# Autodesk Inventor assembly: Finishing_assembly
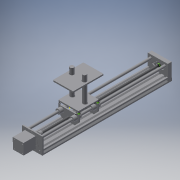
[picture p0: Inventor's stored thumbnail of the model, 180x180]
Saved by Autodesk Inventor 2019 (Build 230136000, 136)
## iProperties
Created: 2021-06-25
Part Number: Finishing_assembly
Document SubType Name: Assembly
Designer: 91742
Author: 91742
## Documents named in this file (17)
- C:\Users\91742\3D Objects\Finishing_assembly.iam
- C:\Users\91742\3D Objects\Rail_finished.ipt
- C:\Users\91742\3D Objects\Stepper_to_rail.ipt
- C:\Users\91742\3D Objects\End_atrail.ipt
- C:\Users\91742\3D Objects\Ball Baering.ipt
- C:\Users\91742\3D Objects\Dampner.ipt
- C:\Users\91742\3D Objects\Motor.ipt
- C:\Users\91742\3D Objects\Coupler.ipt
- C:\Users\91742\3D Objects\Side_rod.ipt
- C:\Users\91742\3D Objects\Steeper nut.ipt
- C:\Users\91742\3D Objects\Part5.ipt
- C:\Users\91742\3D Objects\Threaded rod.ipt
- C:\Users\91742\3D Objects\boltswrew.ipt
- C:\Users\91742\3D Objects\Middle_part.ipt
- C:\Users\91742\3D Objects\Linear_ballbearing.ipt
- C:\Users\91742\3D Objects\Final_mainstage.ipt
- C:\Users\91742\3D Objects\Finished_vertical stage.ipt
## Components (28 placed, 16 different names)
1. Rail_finished:1 — Mate:1, Flush:1, Flush:2, Flush:6
2. Rail_finished:2 — Mate:1, Flush:1, Flush:2, Mate:2, Flush:3, Flush:4, Mate:3, Flush:5
3. Stepper_to_rail:1 — Mate:2, Flush:3, Flush:4, Mate:5, Insert:3, Insert:5, Flush:7, Insert:7, Flush:8, Insert:8, Insert:9, Insert:10, Mate:9, Insert:11
4. End_atrail:1 — Mate:3, Flush:5, Flush:6, Mate:4, Insert:1, Insert:2, Insert:12, Insert:13, Insert:14, Insert:15
5. Ball Baering:1 — Mate:4, Insert:1, Insert:2
6. Dampner:1 — Mate:5, Insert:3, Mate:6, Mate:7, Mate:8, Insert:4, Insert:5
7. Motor:1 — Mate:6, Mate:7, Mate:8, Insert:4, Insert:6
8. Coupler:1 — Insert:6, Insert:16
9. Side_rod:1 — Flush:7, Insert:7, Insert:22, Mate:13
10. Side_rod:2 — Flush:8, Insert:8, Mate:10, Mate:12
11. Steeper nut:1 — Insert:10
12. Steeper nut:2 — Mate:9
13. Steeper nut:3 — Insert:9
14. Steeper nut:4 — Insert:11
15. Part5:1 — Insert:15
16. Part5:2 — Insert:14
17. Part5:3 — Insert:12
18. Part5:4 — Insert:13
19. Threaded rod:1 — Insert:16
20. boltswrew:1 — Insert:21
21. Middle_part:1 — Insert:17, Insert:18, Insert:21, Mate:11, Insert:24
22. Middle_part:2 — Insert:19, Insert:20, Mate:11, Insert:23
23. Linear_ballbearing:1 — Insert:17, Mate:12
24. Linear_ballbearing:2 — Insert:18, Mate:13
25. Linear_ballbearing:3 — Insert:19, Mate:10
26. Linear_ballbearing:4 — Insert:20, Insert:22
27. Final_mainstage:1 — Insert:23, Insert:24, Insert:25, Mate:14
28. Finished_vertical stage:1 — Insert:25, Mate:14
## Relationships (47: Insert 25, Mate 14, Flush 8)
- Mate:1: Rail_finished:1 ↔ Rail_finished:2
- Flush:1: Rail_finished:1 ↔ Rail_finished:2
- Flush:2: Rail_finished:1 ↔ Rail_finished:2
- Mate:2: Rail_finished:2 ↔ Stepper_to_rail:1
- Flush:3: Rail_finished:2 ↔ Stepper_to_rail:1
- Flush:4: Rail_finished:2 ↔ Stepper_to_rail:1
- Mate:3: Rail_finished:2 ↔ End_atrail:1
- Flush:5: Rail_finished:2 ↔ End_atrail:1
- Flush:6: Rail_finished:1 ↔ End_atrail:1
- Mate:4: End_atrail:1 ↔ Ball Baering:1
- Insert:1: End_atrail:1 ↔ Ball Baering:1
- Insert:2: End_atrail:1 ↔ Ball Baering:1
- Mate:5: Stepper_to_rail:1 ↔ Dampner:1
- Insert:3: Stepper_to_rail:1 ↔ Dampner:1
- Mate:6: Dampner:1 ↔ Motor:1
- Mate:7: Dampner:1 ↔ Motor:1
- Mate:8: Dampner:1 ↔ Motor:1
- Insert:4: Dampner:1 ↔ Motor:1
- Insert:5: Stepper_to_rail:1 ↔ Dampner:1
- Insert:6 (-5 mm): Motor:1 ↔ Coupler:1
- Flush:7: Stepper_to_rail:1 ↔ Side_rod:1
- Insert:7: Stepper_to_rail:1 ↔ Side_rod:1
- Flush:8: Stepper_to_rail:1 ↔ Side_rod:2
- Insert:8: Stepper_to_rail:1 ↔ Side_rod:2
- Insert:9: Stepper_to_rail:1 ↔ Steeper nut:3
- Insert:10: Stepper_to_rail:1 ↔ Steeper nut:1
- Mate:9: Stepper_to_rail:1 ↔ Steeper nut:2
- Insert:11: Stepper_to_rail:1 ↔ Steeper nut:4
- Insert:12: End_atrail:1 ↔ Part5:3
- Insert:13: End_atrail:1 ↔ Part5:4
- Insert:14: End_atrail:1 ↔ Part5:2
- Insert:15: End_atrail:1 ↔ Part5:1
- Insert:16: Coupler:1 ↔ Threaded rod:1
- Insert:17 (-15 mm): Middle_part:1 ↔ Linear_ballbearing:1
- Insert:18 (-15 mm): Middle_part:1 ↔ Linear_ballbearing:2
- Insert:19 (-15 mm): Middle_part:2 ↔ Linear_ballbearing:3
- Insert:20 (-15 mm): Middle_part:2 ↔ Linear_ballbearing:4
- Insert:21: boltswrew:1 ↔ Middle_part:1
- Insert:22 (-381 mm): Side_rod:1 ↔ Linear_ballbearing:4
- Mate:10: Side_rod:2 ↔ Linear_ballbearing:3
- Mate:11 (70 mm): Middle_part:1 ↔ Middle_part:2
- Mate:12: Side_rod:2 ↔ Linear_ballbearing:1
- Mate:13: Side_rod:1 ↔ Linear_ballbearing:2
- Insert:23: Middle_part:2 ↔ Final_mainstage:1
- Insert:24: Middle_part:1 ↔ Final_mainstage:1
- Insert:25 (-25 mm): Final_mainstage:1 ↔ Finished_vertical stage:1
- Mate:14: Final_mainstage:1 ↔ Finished_vertical stage:1
